# Autodesk Inventor assembly: __CAVITY_AND_IMAGING_OPTICS__
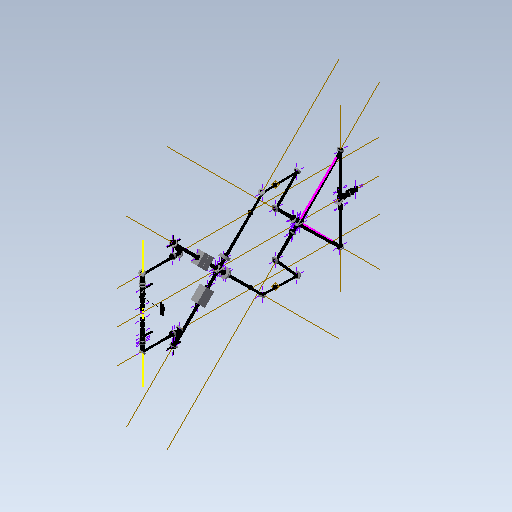
[picture p0: Inventor's stored thumbnail of the model, 512x512]
Saved by Autodesk Inventor 2020 (Build 240168000, 168)
## iProperties
Created: 2016-11-29
Part Number: __CAVITY_AND_IMAGING_OPTICS__
Document SubType Name: Assembly
Designer: map
Author: map
## Documents named in this file (4)
- C:\Users\whgu0532\Documents\4Pi\4Pi-Oxford\__CAVITY_AND_IMAGING_OPTICS__.iam
- C:\Users\whgu0532\Documents\4Pi\4Pi-Oxford\LowerArm__Cavity and Imaging Optics- R8_Old_config0004.iam
- C:\Users\whgu0532\Documents\4Pi\4Pi-Oxford\UpperArm__Cavity and Imaging Optics- R8_Old_config0001.iam
- C:\Users\whgu0532\Documents\4Pi\4Pi-Oxford\__MASTER__.ipt
## Components (3 placed, 3 different names)
1. UpperArm__Cavity and Imaging Optics- R8_Old_config0001:1 [sub-assembly] — Mate:1, Insert:1, Mate:2, Mate:4, Mate:6, Mate:8, Mate:12
2. LowerArm__Cavity and Imaging Optics- R8_Old_config0004:1 [sub-assembly] — Insert:1, Mate:3, Mate:5, Mate:7, Mate:9, Mate:13
3. __MASTER__:1 — Mate:4, Mate:5, Mate:6, Mate:7, Mate:8, Mate:9, Mate:12, Mate:13
## Relationships (12: Mate 11, Insert 1)
- Mate:1: UpperArm__Cavity and Imaging Optics- R8_Old_config0001:1
- Insert:1: UpperArm__Cavity and Imaging Optics- R8_Old_config0001:1 ↔ LowerArm__Cavity and Imaging Optics- R8_Old_config0004:1
- Mate:2: UpperArm__Cavity and Imaging Optics- R8_Old_config0001:1
- Mate:3: LowerArm__Cavity and Imaging Optics- R8_Old_config0004:1
- Mate:4: UpperArm__Cavity and Imaging Optics- R8_Old_config0001:1 ↔ __MASTER__:1
- Mate:5: LowerArm__Cavity and Imaging Optics- R8_Old_config0004:1 ↔ __MASTER__:1
- Mate:6: UpperArm__Cavity and Imaging Optics- R8_Old_config0001:1 ↔ __MASTER__:1
- Mate:7: LowerArm__Cavity and Imaging Optics- R8_Old_config0004:1 ↔ __MASTER__:1
- Mate:8: UpperArm__Cavity and Imaging Optics- R8_Old_config0001:1 ↔ __MASTER__:1
- Mate:9: LowerArm__Cavity and Imaging Optics- R8_Old_config0004:1 ↔ __MASTER__:1
- Mate:12: UpperArm__Cavity and Imaging Optics- R8_Old_config0001:1 ↔ __MASTER__:1
- Mate:13: LowerArm__Cavity and Imaging Optics- R8_Old_config0004:1 ↔ __MASTER__:1
